# Autodesk Inventor assembly: MotorToGear
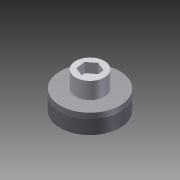
[picture p0: Inventor's stored thumbnail of the model, 180x180]
Saved by Autodesk Inventor 2012 (Build 160160000, 160)
## iProperties
Created: 2011-10-20
Part Number: MotorToGear
Document SubType Name: Assembly
Designer: KuttaA
Author: KuttaA
## Documents named in this file (3)
- C:\Users\KuttaA\Dropbox\Hexapod Research\Leg Design\Other Parts\inter\MotorToGear.iam
- C:\Users\KuttaA\Dropbox\Hexapod Research\Leg Design\Other Parts\inter\NewScrewDrive\Design Accelerator\Spur Gear22.ipt
- C:\Users\KuttaA\Dropbox\Hexapod Research\Leg Design\Other Parts\inter\MotorToGear.ipt
## Components (2 placed, 2 different names)
1. Spur Gear2:1 — Mate:1, Mate:2
2. MotorToGear:1 — Mate:1, Mate:2
## Relationships (2: Mate 2)
- Mate:1: Spur Gear2:1 ↔ MotorToGear:1
- Mate:2: Spur Gear2:1 ↔ MotorToGear:1
